# Autodesk Inventor assembly: Grua Maya.ipt
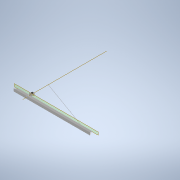
[picture p0: Inventor's stored thumbnail of the model, 180x180]
Saved by Autodesk Inventor 2020 (Build 240168000, 168)
## iProperties
Created: 2019-10-05
Part Number: Grua Maya.ipt
Document SubType Name: Assembly
Designer: dasa1
Author: dasa1
## Documents named in this file (3)
- C:\Users\dasa1\OneDrive\Documents\Inventor\Virtualización Maya\Grua Maya.ipt.iam
- C:\Users\dasa1\OneDrive\Documents\Inventor\Virtualización Maya\Grua Maya.ipt
- C:\Users\dasa1\OneDrive\Documents\Inventor\Virtualización Maya\motor.ipt
## Components (2 placed, 2 different names)
1. Grua Maya:1 — Nivelación:1, Ángulo:1, Coincidencia:1, Nivelación:2, Nivelación:3
2. motor:1 — Ángulo:1, Coincidencia:1, Nivelación:2, Nivelación:3
## Relationships (5: Flush 3, Angle 1, Mate 1)
- Nivelación:1 [Flush] (35 mm): Grua Maya:1
- Ángulo:1 [Angle] (0 deg): Grua Maya:1 ↔ motor:1
- Coincidencia:1 [Mate]: Grua Maya:1 ↔ motor:1
- Nivelación:2 [Flush]: Grua Maya:1 ↔ motor:1
- Nivelación:3 [Flush] (-65 mm): Grua Maya:1 ↔ motor:1
